# Autodesk Inventor assembly: ChargingConnectorFemale
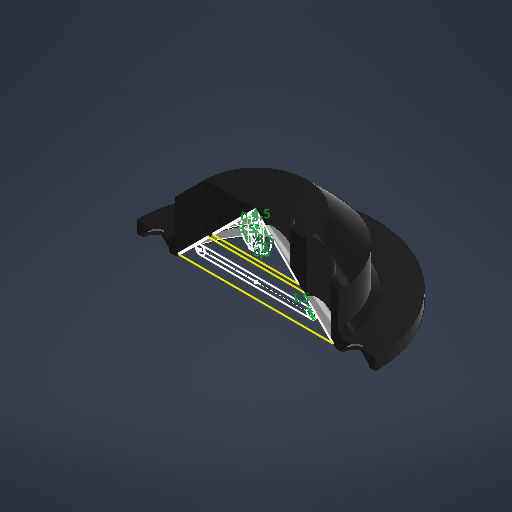
[picture p0: Inventor's stored thumbnail of the model, 512x512]
Saved by Autodesk Inventor 2025 (Build 290162000, 162)
## iProperties
Created: 2025-01-24
Part Number: ChargingConnectorFemale
Document SubType Name: Assembly
Designer: khrip
Author: khrip
## Documents named in this file (4)
- H:\Potamon\3Dmodels\ChargingStation\ChargingConnectorFemale.iam
- H:\Potamon\3Dmodels\ChargingStation\Kathode.ipt
- H:\Potamon\3Dmodels\ChargingStation\Anode.ipt
- H:\Potamon\3Dmodels\ChargingStation\Casing.ipt
## Components (3 placed, 3 different names)
1. Kathode:1
2. Anode:1 — Заподлицо:1
3. Casing:1 — Заподлицо:2
## Relationships (2: Flush 2)
- Заподлицо:1 [Flush]: Anode:1
- Заподлицо:2 [Flush]: Casing:1
